# Autodesk Inventor assembly: Ensamble_Modelo_6R
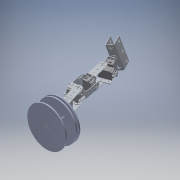
[picture p0: Inventor's stored thumbnail of the model, 180x180]
Saved by Autodesk Inventor 2017 (Build 210142000, 142)
## iProperties
Part Number: Ensamble_Modelo_6R
Material: Genérico
Document SubType Name: Assembly
Designer: Daniel Caycedo
Author: Daniel Caycedo
## Documents named in this file (8)
- C:\Users\Daniel Caycedo\Documents\Daniel SCR\Universidad\Proyecto ingenieria\Modelo_6R\Inventor\Ensamble_Modelo_6R.iam
- C:\Users\Daniel Caycedo\Documents\Daniel SCR\Universidad\Proyecto ingenieria\Modelo_6R\Inventor\Base\Base_modelo_6R.ipt
- C:\Users\Daniel Caycedo\Documents\Daniel SCR\Universidad\Proyecto ingenieria\Modelo_6R\Inventor\Joint_1\Joint_1_modelo_6R.ipt
- C:\Users\Daniel Caycedo\Documents\Daniel SCR\Universidad\Proyecto ingenieria\Modelo_6R\Inventor\Joint_3\Joint_3_modelo_6R.ipt
- C:\Users\Daniel Caycedo\Documents\Daniel SCR\Universidad\Proyecto ingenieria\Modelo_6R\Inventor\Joint_4\Joint_4_modelo_6R.ipt
- C:\Users\Daniel Caycedo\Documents\Daniel SCR\Universidad\Proyecto ingenieria\Modelo_6R\Inventor\Joint_2\Joint_2_modelo_6R.ipt
- C:\Users\Daniel Caycedo\Documents\Daniel SCR\Universidad\Proyecto ingenieria\Modelo_6R\Inventor\Joint_5\Joint_5_modelo_6R.ipt
- C:\Users\Daniel Caycedo\Documents\Daniel SCR\Universidad\Proyecto ingenieria\Modelo_6R\Inventor\Gripper\Servo Bracket - Long U_D‚faut.ipt
## Components (7 placed, 7 different names)
1. Base_modelo_6R:1 — Coincidencia:1, Coincidencia:2
2. Joint_1_modelo_6R:1 — Coincidencia:1, Coincidencia:2, Coincidencia:3, Coincidencia:4
3. Joint_3_modelo_6R:1 — Coincidencia:5, Coincidencia:6, Coincidencia:7, Coincidencia:8
4. Joint_4_modelo_6R:1 — Coincidencia:7, Coincidencia:8, Coincidencia:9, Coincidencia:10
5. Joint_2_modelo_6R:1 — Coincidencia:3, Coincidencia:4, Coincidencia:5, Coincidencia:6
6. Joint_5_modelo_6R:1 — Coincidencia:9, Coincidencia:10, Coincidencia:11, Coincidencia:12
7. Servo Bracket - Long U_D‚faut:1 — Coincidencia:11, Coincidencia:12
## Relationships (12: Mate 12)
- Coincidencia:1 [Mate]: Base_modelo_6R:1 ↔ Joint_1_modelo_6R:1
- Coincidencia:2 [Mate]: Base_modelo_6R:1 ↔ Joint_1_modelo_6R:1
- Coincidencia:3 [Mate]: Joint_1_modelo_6R:1 ↔ Joint_2_modelo_6R:1
- Coincidencia:4 [Mate]: Joint_1_modelo_6R:1 ↔ Joint_2_modelo_6R:1
- Coincidencia:5 [Mate]: Joint_3_modelo_6R:1 ↔ Joint_2_modelo_6R:1
- Coincidencia:6 [Mate]: Joint_3_modelo_6R:1 ↔ Joint_2_modelo_6R:1
- Coincidencia:7 [Mate]: Joint_3_modelo_6R:1 ↔ Joint_4_modelo_6R:1
- Coincidencia:8 [Mate]: Joint_3_modelo_6R:1 ↔ Joint_4_modelo_6R:1
- Coincidencia:9 [Mate]: Joint_4_modelo_6R:1 ↔ Joint_5_modelo_6R:1
- Coincidencia:10 [Mate]: Joint_4_modelo_6R:1 ↔ Joint_5_modelo_6R:1
- Coincidencia:11 [Mate]: Joint_5_modelo_6R:1 ↔ Servo Bracket - Long U_D‚faut:1
- Coincidencia:12 [Mate]: Joint_5_modelo_6R:1 ↔ Servo Bracket - Long U_D‚faut:1
